# Autodesk Inventor assembly: REV-41-1267
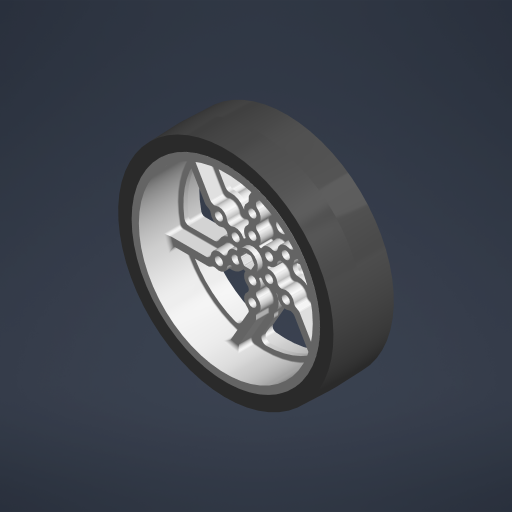
[picture p0: Inventor's stored thumbnail of the model, 512x512]
Saved by Autodesk Inventor 2023 (Build 270158000, 158)
## iProperties
Created: 2018-05-09
Part Number: REV-41-1267
Description: STEP AP214
Document SubType Name: Assembly
Designer: izack
Title: REV-41-1267.STEP
Revision Number: ANY
Sending System: SolidWorks 2017
Preprocessor: SwSTEP 2.0
## Documents named in this file (4)
- D:\Robotics\Custom-Modules-CAD\SwerveDrive V2\SwerveDrive V2 Parts\90mm Grip WheelREV-41-1267 (1).iam
- 90mm Grip Wheel.iam
- D:\Robotics\Custom-Modules-CAD\SwerveDrive V2\SwerveDrive V2 Parts\90mm Grip Wheel90 mm not stealth wheels.ipt
- D:\Robotics\Custom-Modules-CAD\SwerveDrive V2\SwerveDrive V2 Parts\90mm Grip Wheeltread.ipt
## Components (2 placed, 2 different names)
1. 90 mm not stealth wheels_1 — Mate:1, Flush:1, Mate:2
2. tread_2 — Mate:1, Flush:1, Mate:2
## Relationships (3: Mate 2, Flush 1)
- Mate:1: 90 mm not stealth wheels_1 ↔ tread_2
- Flush:1: 90 mm not stealth wheels_1 ↔ tread_2
- Mate:2: 90 mm not stealth wheels_1 ↔ tread_2
